# Autodesk Inventor assembly: ColdStorageCasing
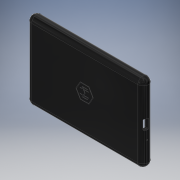
[picture p0: Inventor's stored thumbnail of the model, 180x180]
Saved by Autodesk Inventor 2017 (Build 210142000, 142)
## iProperties
Created: 2018-08-04
Part Number: ColdStorageCasing
Document SubType Name: Assembly
Designer: intelsath
Author: intelsath
## Documents named in this file (4)
- C:\Users\intelsath\Documents\Inventor\Cryptowallet\ColdStorageCasing.iam
- C:\Users\intelsath\Documents\Inventor\Cryptowallet\Casing (Back).ipt
- C:\Users\intelsath\Documents\Inventor\Cryptowallet\LCD+Cover.ipt
- C:\Users\intelsath\Documents\Inventor\Cryptowallet\Button Cap.ipt
## Components (3 placed, 3 different names)
1. Casing (Back):1 — Mate:1, Mate:2, Mate:3, Mate:4, Mate:5, Flush:1, Flush:2, Flush:3, Mate:6
2. LCD+Cover:1 — Mate:1, Mate:2, Mate:3
3. Button Cap:1 — Mate:4, Mate:5, Mate:6
## Relationships (9: Mate 6, Flush 3)
- Mate:1: Casing (Back):1 ↔ LCD+Cover:1
- Mate:2: Casing (Back):1 ↔ LCD+Cover:1
- Mate:3: Casing (Back):1 ↔ LCD+Cover:1
- Mate:4: Casing (Back):1 ↔ Button Cap:1
- Mate:5: Casing (Back):1 ↔ Button Cap:1
- Flush:1: Casing (Back):1
- Flush:2: Casing (Back):1
- Flush:3: Casing (Back):1
- Mate:6 (0.5 mm): Casing (Back):1 ↔ Button Cap:1
